# Autodesk Inventor assembly: Inset Hinge Split Dowel Cup Knock-In T18
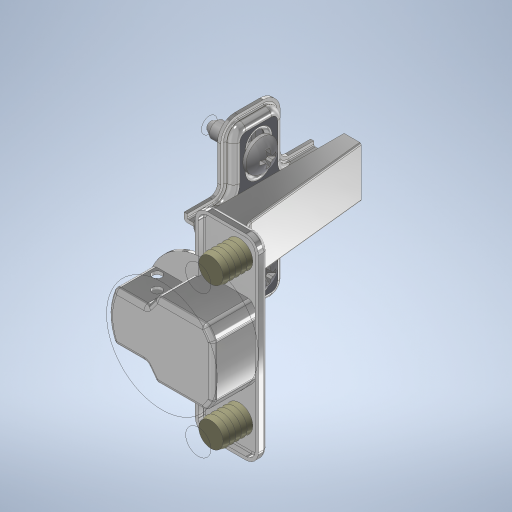
[picture p0: Inventor's stored thumbnail of the model, 512x512]
Saved by Autodesk Inventor 2024 (Build 280153000, 153)
## iProperties
Created: 2013-11-24
Part Number: Inset Hinge Split Dowel Cup Knock-In T18
Document SubType Name: Assembly
Designer: SauliusD
Author: SauliusD
## Documents named in this file (8)
- C:\W4INV 2024 Design\LIBRARY\Hinges\CONCEALED HINGE\Inset Hinge Split Dowel Cup Knock-In T18.iam
- C:\W4INV 2022 Design\LIBRARY\Hinges\Parts\Concelead Hinge\Hinge.ipt
- C:\W4INV 2024 Design\LIBRARY\Hinges\Parts\Concelead Hinge\Lever 1.ipt
- C:\W4INV 2024 Design\LIBRARY\Hinges\Parts\Concelead Hinge\Lever 2.ipt
- C:\W4INV 2022 Design\LIBRARY\Hinges\Parts\Concelead Hinge\Cup.ipt
- C:\W4INV 2024 Design\LIBRARY\Hinges\Parts\Concelead Hinge\Cup\Hinge cup Knock-In.ipt
- C:\W4INV 2024 Design\LIBRARY\Hinges\CONCEALED HINGE.iam
- C:\W4INV 2024 Design\LIBRARY\Hinges\Parts\Concelead Hinge\Hinge\Inset Hinge Split Dowel.ipt
## Components (4 placed, 4 different names)
1. Inset Hinge Split Dowel:1 — Mate:1, Flush:1, Mate:2, Flush:2, Flush:3, Flush:4, Flush:5, Flush:6, Angle:1
2. Lever 1:1 — Flush:1, Mate:2, Mate:4
3. Lever 2:1 — Mate:1, Flush:5, Mate:3
4. Hinge cup Knock-In:1 — Flush:6, Mate:3, Mate:4, Angle:1
## Relationships (11: Flush 6, Mate 4, Angle 1)
- Mate:1: Inset Hinge Split Dowel:1 ↔ Lever 2:1
- Flush:1: Inset Hinge Split Dowel:1 ↔ Lever 1:1
- Mate:2: Inset Hinge Split Dowel:1 ↔ Lever 1:1
- Flush:2: Inset Hinge Split Dowel:1
- Flush:3: Inset Hinge Split Dowel:1
- Flush:4: Inset Hinge Split Dowel:1
- Flush:5: Inset Hinge Split Dowel:1 ↔ Lever 2:1
- Flush:6: Inset Hinge Split Dowel:1 ↔ Hinge cup Knock-In:1
- Mate:3: Lever 2:1 ↔ Hinge cup Knock-In:1
- Mate:4: Lever 1:1 ↔ Hinge cup Knock-In:1
- Angle:1 (90 deg): Inset Hinge Split Dowel:1 ↔ Hinge cup Knock-In:1
